# Autodesk Inventor assembly: 2 rooms side by side
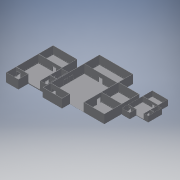
[picture p0: Inventor's stored thumbnail of the model, 180x180]
Saved by Autodesk Inventor 2017 (Build 210142000, 142)
## iProperties
Created: 2018-05-03
Part Number: 2 rooms side by side
Document SubType Name: Assembly
Designer: braxtonwright
Author: braxtonwright
## Documents named in this file (4)
- D:\School\Game develpment\geoscape\helping\2 rooms side by side.iam
- D:\School\Game develpment\geoscape\helping\second floor down for landon.ipt
- C:\Users\braxtonwright\Documents\GitHub\Geoscape\Blender Team\Landon's work\Top Office Layer part 1.ipt
- D:\School\Game develpment\geoscape\helping\second floor down for landon scaled.ipt
## Components (3 placed, 3 different names)
1. second floor down for landon:1 — Flush:1, Mate:1
2. Top Office Layer part 1:1 — Flush:1, Mate:1, Mate:2, Flush:2
3. second floor down for landon scaled:1 — Mate:2, Flush:2
## Relationships (4: Flush 2, Mate 2)
- Flush:1: second floor down for landon:1 ↔ Top Office Layer part 1:1
- Mate:1 (25.4 mm): second floor down for landon:1 ↔ Top Office Layer part 1:1
- Mate:2 (25.4 mm): Top Office Layer part 1:1 ↔ second floor down for landon scaled:1
- Flush:2: Top Office Layer part 1:1 ↔ second floor down for landon scaled:1
